# Autodesk Inventor assembly: AUT_60GHz_Horn_Mounted
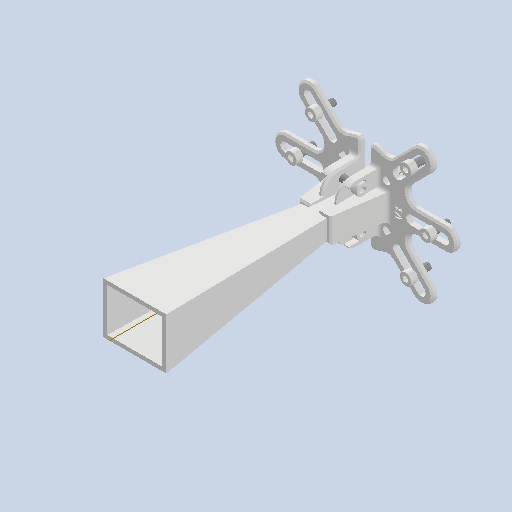
[picture p0: Inventor's stored thumbnail of the model, 512x512]
Saved by Autodesk Inventor 2023.2 (Build 272271000, 271)
## iProperties
Created: 2024-07-01
Part Number: AUT_60GHz_Horn_Mounted
Document SubType Name: Assembly
Designer: Nils Bade
Author: Nils Bade
## Documents named in this file (6)
- C:\Users\nilsb\Documents\Inventor\Projektarbeit-Bade\AUT-Mountings\AUT_60GHz_Horn_Mounted.iam
- C:\Users\nilsb\Documents\Inventor\Projektarbeit-Bade\AUT-Mountings\AUT_60GHz_HornDummy.ipt
- C:\Users\nilsb\Documents\Inventor\Projektarbeit-Bade\AUT-Mountings\AUT_MOUNT_60GHz_Hornantenna.ipt
- C:\Users\nilsb\Documents\Inventor\Projektarbeit-Bade\Schrauben\Cap Head Screw M4x12 - DIN912.ipt
- C:\Users\nilsb\Documents\Inventor\Projektarbeit-Bade\RatRig_Standards\Hex Nut - M4 DIN934.ipt
- C:\Users\nilsb\Documents\Inventor\Projektarbeit-Bade\Schrauben\Cap Head Screw M4x10 - DIN912.ipt
## Components (13 placed, 5 different names)
1. AUT_60GHz_HornDummy:1 — Passend:3, Passend:4, Passend:5, Passend:6
2. 60GHz_Hornantenna_mount_V1:3 — Passend:1, Passend:2, Passend:4, Passend:5, Passend:6, Winkel:1, Winkel:2, Passend:13, Passend:14
3. 60GHz_Hornantenna_mount_V1:4 — Passend:1, Passend:2, Passend:3, Passend:7, Passend:8, Passend:9, Passend:10, Passend:17
4. Cap Head Screw M4x12 - DIN912:1 — Passend:7, Passend:10, Passend:11
5. Cap Head Screw M4x12 - DIN912:2 — Passend:8, Passend:9, Passend:12
6. Hex Nut - M4 DIN934:1 — Passend:11, Winkel:2, Passend:13
7. Hex Nut - M4 DIN934:2 — Passend:12, Winkel:1, Passend:14
8. Cap Head Screw M4x10 - DIN912:1 — Passend:15, Passend:16, Passend:17
9. Cap Head Screw M4x10 - DIN912:2
10. Cap Head Screw M4x10 - DIN912:4
11. Cap Head Screw M4x10 - DIN912:5
12. Cap Head Screw M4x10 - DIN912:6
13. Cap Head Screw M4x10 - DIN912:8
## Component patterns: (8 elements, first: Cap Head Screw M4x10 - DIN912:1)
## Relationships (19: Mate 17, Angle 2)
- Passend:1 [Mate]: 60GHz_Hornantenna_mount_V1:3 ↔ 60GHz_Hornantenna_mount_V1:4
- Passend:2 [Mate]: 60GHz_Hornantenna_mount_V1:3 ↔ 60GHz_Hornantenna_mount_V1:4
- Passend:3 [Mate]: AUT_60GHz_HornDummy:1 ↔ 60GHz_Hornantenna_mount_V1:4
- Passend:4 [Mate]: AUT_60GHz_HornDummy:1 ↔ 60GHz_Hornantenna_mount_V1:3
- Passend:5 [Mate]: AUT_60GHz_HornDummy:1 ↔ 60GHz_Hornantenna_mount_V1:3
- Passend:6 [Mate]: AUT_60GHz_HornDummy:1 ↔ 60GHz_Hornantenna_mount_V1:3
- Passend:7 [Mate]: 60GHz_Hornantenna_mount_V1:4 ↔ Cap Head Screw M4x12 - DIN912:1
- Passend:8 [Mate]: 60GHz_Hornantenna_mount_V1:4 ↔ Cap Head Screw M4x12 - DIN912:2
- Passend:9 [Mate]: 60GHz_Hornantenna_mount_V1:4 ↔ Cap Head Screw M4x12 - DIN912:2
- Passend:10 [Mate]: 60GHz_Hornantenna_mount_V1:4 ↔ Cap Head Screw M4x12 - DIN912:1
- Passend:11 [Mate]: Cap Head Screw M4x12 - DIN912:1 ↔ Hex Nut - M4 DIN934:1
- Passend:12 [Mate]: Cap Head Screw M4x12 - DIN912:2 ↔ Hex Nut - M4 DIN934:2
- Winkel:1 [Angle] (0 deg): 60GHz_Hornantenna_mount_V1:3 ↔ Hex Nut - M4 DIN934:2
- Winkel:2 [Angle] (0 deg): 60GHz_Hornantenna_mount_V1:3 ↔ Hex Nut - M4 DIN934:1
- Passend:13 [Mate]: 60GHz_Hornantenna_mount_V1:3 ↔ Hex Nut - M4 DIN934:1
- Passend:14 [Mate]: 60GHz_Hornantenna_mount_V1:3 ↔ Hex Nut - M4 DIN934:2
- Passend:15 [Mate] (40 mm): Cap Head Screw M4x10 - DIN912:1
- Passend:16 [Mate]: Cap Head Screw M4x10 - DIN912:1
- Passend:17 [Mate]: 60GHz_Hornantenna_mount_V1:4 ↔ Cap Head Screw M4x10 - DIN912:1
